# Autodesk Inventor assembly: Assemblies_Cradle
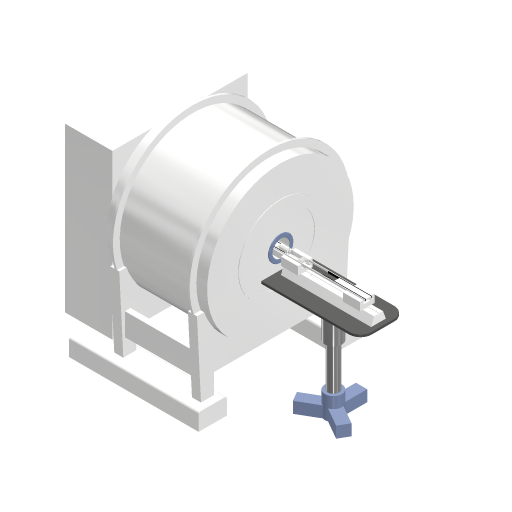
[picture p0: Inventor's stored thumbnail of the model, 512x512]
Saved by Autodesk Inventor 2024 (Build 280153000, 153)
## iProperties
Created: 2021-10-08
Part Number: Assemblies_Cradle
Document SubType Name: Assembly
Designer: Rik Ubaghs
Author: Rik Ubaghs
## Documents named in this file (12)
- C:\Users\Rik\Desktop\open_mr_cradle_mouse\production\ipt\assemblies\assemblies_complete.iam
- C:\Users\Rik\Desktop\open_mr_cradle_mouse\production\ipt\cradle\cradle_slide_front_mk1.ipt
- C:\Users\Rik\Desktop\open_mr_cradle_mouse\production\ipt\cradle\cradle_slidebase_mk1.ipt
- C:\Users\Rik\Desktop\open_mr_cradle_mouse\production\ipt\cradle\cradle_av4m_ext.ipt
- C:\Users\Rik\Desktop\open_mr_cradle_mouse\production\ipt\cradle\cradle_c1515m_ext.ipt
- C:\Users\Rik\Desktop\open_mr_cradle_mouse\production\ipt\cradle\cradle_mb1015m_ext.ipt
- C:\Users\Rik\Desktop\open_mr_cradle_mouse\production\ipt\cradle\cradle_p300m_ext.ipt
- C:\Users\Rik\Desktop\open_mr_cradle_mouse\production\ipt\cradle\cradle_pb4m_ext.ipt
- C:\Users\Rik\Desktop\open_mr_cradle_mouse\production\ipt\cradle\cradle_slide_back_mk1.ipt
- C:\Users\Rik\Desktop\open_mr_cradle_mouse\production\ipt\cradle\cradle_psham_ext.ipt
- C:\Users\Rik\Desktop\open_mr_cradle_mouse\production\ipt\assemblies\assemblies_cradle.iam
- C:\Users\Rik\Desktop\open_mr_cradle_mouse\production\ipt\assemblies\assemblies_mri.iam
## Components (17 placed, 11 different names)
1. assemblies_mri:1 [sub-assembly] — Mate:129, Mate:130, Flush:25, Mate:131
2. assemblies_cradle:1 [sub-assembly] — Mate:233, Mate:234, Mate:235, Flush:43
3. cradle_av4m_ext:1
4. cradle_av4m_ext:2 — Mate:131
5. cradle_av4m_ext:3
6. cradle_av4m_ext:4
7. cradle_c1515m_ext:1
8. cradle_mb1015m_ext:1
9. cradle_mb1015m_ext:2
10. cradle_p300m_ext:1
11. cradle_pb4m_ext:1
12. cradle_psham_ext:1
13. cradle_slidebase_mk1:1 — Mate:129, Mate:130
14. cradle_slidebase_mk1:2
15. cradle_slide_back_mk1:1 — Mate:235
16. cradle_slide_back_mk1:2 — Mate:233, Mate:234
17. cradle_slide_front_mk1:1 — Flush:25, Flush:43
## Relationships (44: Mate 30, Flush 9, Tangent 3, Angle 2)
- [Mate]: cradle_slidebase_mk1:1 ↔ cradle_slide_back_mk1:2
- [Mate]: cradle_slidebase_mk1:1 ↔ cradle_slide_back_mk1:2
- [Mate]: cradle_slidebase_mk1:1 ↔ cradle_slide_back_mk1:2
- [Mate]: cradle_slidebase_mk1:2 ↔ cradle_slide_front_mk1:1
- [Mate]: cradle_slidebase_mk1:2 ↔ cradle_slide_front_mk1:1
- [Mate]: cradle_slidebase_mk1:2 ↔ cradle_slide_front_mk1:1
- [Mate]: cradle_p300m_ext:1 ↔ cradle_pb4m_ext:1
- [Mate]: cradle_mb1015m_ext:1 ↔ cradle_pb4m_ext:1
- [Mate]: cradle_av4m_ext:2 ↔ cradle_mb1015m_ext:1
- [Mate]: cradle_av4m_ext:4 ↔ cradle_mb1015m_ext:1
- [Mate]: cradle_av4m_ext:4 ↔ cradle_mb1015m_ext:1
- [Mate]: cradle_av4m_ext:2 ↔ cradle_mb1015m_ext:1
- [Mate]: cradle_av4m_ext:1 ↔ cradle_mb1015m_ext:1
- [Mate]: cradle_av4m_ext:3 ↔ cradle_mb1015m_ext:1
- [Mate]: cradle_av4m_ext:3 ↔ cradle_mb1015m_ext:1
- [Mate]: cradle_av4m_ext:1 ↔ cradle_mb1015m_ext:1
- [Mate]: cradle_c1515m_ext:1 ↔ cradle_p300m_ext:1
- [Angle] (0 deg): cradle_c1515m_ext:1 ↔ cradle_mb1015m_ext:1
- [Tangent]: cradle_c1515m_ext:1 ↔ cradle_mb1015m_ext:2
- [Mate]: cradle_c1515m_ext:1 ↔ cradle_mb1015m_ext:2
- [Angle] (0 deg): cradle_c1515m_ext:1 ↔ cradle_mb1015m_ext:2
- [Flush] (-10 mm): cradle_c1515m_ext:1 ↔ cradle_mb1015m_ext:2
- [Mate]: cradle_p300m_ext:1 ↔ cradle_pb4m_ext:1
- [Tangent] (2 mm): cradle_mb1015m_ext:1 ↔ cradle_pb4m_ext:1
- [Tangent] (27 mm): cradle_mb1015m_ext:1 ↔ cradle_pb4m_ext:1
- [Flush]: cradle_slide_back_mk1:2 ↔ cradle_slide_front_mk1:1
- [Flush]: cradle_slidebase_mk1:1 ↔ cradle_slidebase_mk1:2
- [Mate] (400 mm): cradle_slide_back_mk1:2 ↔ cradle_slide_front_mk1:1
- [Flush]: cradle_slide_back_mk1:1 ↔ cradle_slide_back_mk1:2
- [Flush]: cradle_slide_back_mk1:1 ↔ cradle_slide_back_mk1:2
- [Mate]: cradle_mb1015m_ext:2 ↔ cradle_slide_back_mk1:1
- [Flush] (-10 mm): cradle_mb1015m_ext:2 ↔ cradle_slide_back_mk1:1
- [Flush] (20 mm): cradle_mb1015m_ext:2 ↔ cradle_slide_back_mk1:1
- [Mate]: cradle_c1515m_ext:1 ↔ cradle_psham_ext:1
- [Mate]: cradle_p300m_ext:1 ↔ cradle_psham_ext:1
- [Mate]: cradle_pb4m_ext:1 ↔ cradle_psham_ext:1
- Mate:129: assemblies_mri:1 ↔ cradle_slidebase_mk1:1
- Mate:130: assemblies_mri:1 ↔ cradle_slidebase_mk1:1
- Flush:25: assemblies_mri:1 ↔ cradle_slide_front_mk1:1
- Mate:131: assemblies_mri:1 ↔ cradle_av4m_ext:2
- Mate:233 (1 mm): assemblies_cradle:1 ↔ cradle_slide_back_mk1:2
- Mate:234: assemblies_cradle:1 ↔ cradle_slide_back_mk1:2
- Mate:235 (1 mm): assemblies_cradle:1 ↔ cradle_slide_back_mk1:1
- Flush:43: assemblies_cradle:1 ↔ cradle_slide_front_mk1:1
